# Autodesk Inventor assembly: Montagem1
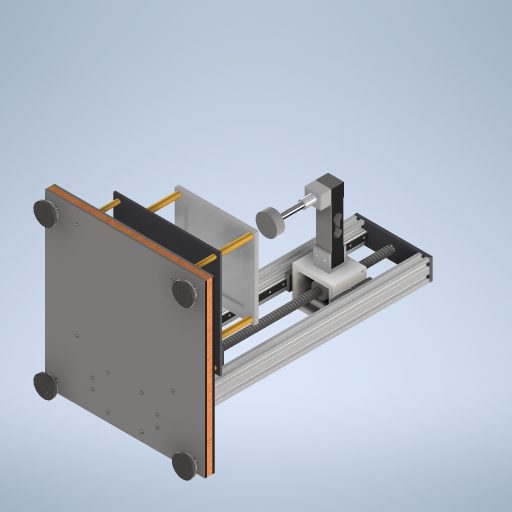
[picture p0: Inventor's stored thumbnail of the model, 512x512]
Saved by Autodesk Inventor 2023 (Build 270158000, 158)
## iProperties
Created: 2023-03-18
Part Number: Montagem1
Document SubType Name: Assembly
Designer: Mateus
Mass: 15449.6 g
Surface Area: 13309.4 cm^2
Volume: 3131.3 cm^3
Density: 4.93393 g/cm^3
Author: Mateus
## Documents named in this file (35)
- C:\Users\Mateus PC\OneDrive\TCC\Desenho 3D\Montagem1.iam
- C:\Users\Mateus PC\OneDrive\TCC\Desenho 3D\Base.ipt
- C:\Users\Mateus PC\OneDrive\TCC\Desenho 3D\Fuso.ipt
- C:\Users\Mateus PC\OneDrive\TCC\Desenho 3D\Motor.ipt
- C:\Users\Mateus PC\OneDrive\TCC\Desenho 3D\Suporte 1.ipt
- C:\Users\Mateus PC\OneDrive\TCC\Desenho 3D\Espaçador 1.ipt
- C:\Users\Mateus PC\OneDrive\TCC\Desenho 3D\Espaçador 2.ipt
- C:\Users\Mateus PC\OneDrive\TCC\Desenho 3D\Suporte 2.ipt
- C:\Users\Mateus PC\OneDrive\TCC\Desenho 3D\Contra ponto.ipt
- C:\Users\Mateus PC\OneDrive\TCC\Desenho 3D\Espaçador 3.ipt
- C:\Users\Mateus PC\OneDrive\TCC\Desenho 3D\Mesa 1.ipt
- C:\Users\Mateus PC\OneDrive\TCC\Desenho 3D\Guia.ipt
- C:\Users\Mateus PC\OneDrive\TCC\Desenho 3D\Suporte guia.ipt
- C:\Users\Mateus PC\OneDrive\TCC\Desenho 3D\Guia trilho.ipt
- C:\Users\Mateus PC\OneDrive\TCC\Desenho 3D\Lado caixa 1.ipt
- C:\Users\Mateus PC\OneDrive\TCC\Desenho 3D\Lado caixa 2.ipt
- C:\Users\Mateus PC\OneDrive\TCC\Desenho 3D\Célula de carga 2.ipt
- C:\Users\Mateus PC\OneDrive\TCC\Desenho 3D\Suporte braço 2.0.ipt
- C:\Users\Mateus PC\OneDrive\TCC\Desenho 3D\Suporte ponta.ipt
- C:\Users\Mateus PC\OneDrive\TCC\Desenho 3D\Trilho 2.ipt
- C:\Users\Mateus PC\OneDrive\TCC\Desenho 3D\Mesa 2.ipt
- C:\Users\Mateus PC\OneDrive\TCC\Desenho 3D\Espaçador 4.ipt
- C:\Users\Mateus PC\OneDrive\TCC\Desenho 3D\Mesa 3.ipt
- C:\Users\Mateus PC\OneDrive\TCC\Desenho 3D\Suporte mesa.ipt
- C:\Users\Mateus PC\OneDrive\TCC\Desenho 3D\Probe.ipt
- C:\Users\Mateus PC\OneDrive\TCC\Desenho 3D\Base madeira.ipt
- C:\Users\Mateus PC\OneDrive\TCC\Desenho 3D\Perfil aluminio 2.ipt
- C:\Users\Mateus PC\OneDrive\TCC\Desenho 3D\Lado caixa 3.ipt
- C:\Users\Mateus PC\OneDrive\TCC\Desenho 3D\Pés.ipt
- C:\Users\Mateus PC\OneDrive\TCC\Desenho 3D\Montagem1\AIP\FEA\eaa23tyn4.fins
- C:\Users\Mateus PC\OneDrive\TCC\Desenho 3D\Montagem1\AIP\FEA\eaa23tyo0.fsat
- C:\Users\Mateus PC\OneDrive\TCC\Desenho 3D\Montagem1\AIP\FEA\eaa23tyo0.ftes
- C:\Users\Mateus PC\OneDrive\TCC\Desenho 3D\Montagem1\AIP\FEA\eaa23tyo0.fwiz
- C:\Users\Mateus PC\OneDrive\TCC\Desenho 3D\Montagem1\AIP\FEA\eaa23tytc.fmsh
- C:\Users\Mateus PC\OneDrive\TCC\Desenho 3D\Montagem1\AIP\FEA\eaa23tytd.fres
## Components (51 placed, 28 different names)
1. Base:1 — Coincidente:13, Alinhado:11, Coincidente:17, Alinhado:12, Coincidente:27, Coincidente:28, Coincidente:29, Coincidente:30, Coincidente:48, Alinhado:28, Alinhado:29, Coincidente:269, Alinhado:84, Coincidente:273, Alinhado:86, Coincidente:275, Flush:104
2. Fuso:1 — Coincidente:9, Coincidente:10, Coincidente:13, Coincidente:49, Coincidente:248, Mate:285
3. Motor:1 — Coincidente:9, Coincidente:10, Alinhado:11, Coincidente:24, Coincidente:25, Coincidente:26, Coincidente:40
4. Suporte 1:1 — Coincidente:24, Coincidente:25, Coincidente:26, Coincidente:31, Coincidente:32, Coincidente:33, Coincidente:34, Coincidente:35, Coincidente:36, Coincidente:37, Coincidente:38, Coincidente:39, Alinhado:22, Mate:117
5. Espaçador 1:1 — Coincidente:29, Coincidente:34, Mate:117
6. Espaçador 1:2 — Coincidente:27, Coincidente:33
7. Espaçador 1:3 — Coincidente:30, Coincidente:32
8. Espaçador 1:4 — Coincidente:28, Coincidente:31
9. Espaçador 2:1 — Coincidente:35, Alinhado:19, Alinhado:20, Coincidente:39, Coincidente:41
10. Espaçador 2:2 — Coincidente:36, Alinhado:20, Alinhado:21
11. Espaçador 2:3 — Coincidente:38, Alinhado:19
12. Espaçador 2:4 — Coincidente:37, Alinhado:21
13. Suporte 2:1 — Coincidente:40, Alinhado:22, Coincidente:41
14. Contra ponto:1 — Coincidente:248, Alinhado:91, Coincidente:278
15. Espaçador 3:1 — Coincidente:45, Alinhado:25, Alinhado:26
16. Espaçador 3:2 — Alinhado:25, Coincidente:47, Coincidente:48, Mate:119
17. Espaçador 3:3 — Coincidente:44, Alinhado:27
18. Espaçador 3:4 — Coincidente:43, Alinhado:26, Alinhado:27
19. Mesa 1:1 — Coincidente:43, Coincidente:44, Coincidente:45, Coincidente:47, Alinhado:28, Alinhado:29, Alinhado:61, Alinhado:62, Mate:119, Mate:121
20. Guia:1 — Coincidente:49, Coincidente:50, Coincidente:51
21. Suporte guia:1 — Coincidente:50, Coincidente:51, Mate:284, Flush:100
22. Guia trilho:1 — Mate:60, Coincidente:206, Alinhado:74
23. Guia trilho:2 — Mate:60, Flush:30, Coincidente:205, Alinhado:74, Alinhado:75, Coincidente:208, Mate:279
24. Guia trilho:3 — Mate:61, Alinhado:72, Alinhado:73
25. Guia trilho:4 — Mate:61, Flush:30, Alinhado:72, Alinhado:73, Coincidente:204, Alinhado:75, Mate:280, Flush:99
26. Lado caixa 1:2 — Mate:115, Flush:65, Coincidente:126, Flush:96, Flush:97, Mate:283
27. Lado caixa 2:2 — Flush:94, Flush:95, Mate:281, Mate:282, Mate:284, Flush:100
28. Célula de carga 2:1 — Coincidente:98, Alinhado:56, Alinhado:57, Flush:63, Flush:64, Mate:114
29. Suporte braço 2.0:1 — Flush:63, Flush:64, Mate:114, Mate:115, Flush:65, Coincidente:126
30. Suporte ponta:1 — Coincidente:98, Alinhado:56, Alinhado:57, Coincidente:270, Coincidente:271
31. Trilho 2:1 — Alinhado:58, Alinhado:59, Coincidente:205, Coincidente:206, Coincidente:208, Coincidente:269, Coincidente:276
32. Trilho 2:2 — Alinhado:58, Alinhado:59, Coincidente:204, Coincidente:277, Alinhado:90
33. Mesa 2:1 — Coincidente:106, Coincidente:107, Coincidente:108, Coincidente:109, Coincidente:110, Alinhado:61, Alinhado:62, Coincidente:111, Coincidente:112, Coincidente:113
34. Espaçador 4:1 — Coincidente:108, Flush:67, Flush:68, Mate:125
35. Espaçador 4:2 — Coincidente:106, Coincidente:110, Flush:68, Mate:123, Mate:124
36. Espaçador 4:3 — Coincidente:109, Flush:66, Flush:67
37. Espaçador 4:4 — Coincidente:107, Flush:66, Mate:122
38. Mesa 3:1 — Coincidente:111, Coincidente:112, Coincidente:113
39. Suporte mesa:1 — Flush:69, Flush:70, Mate:121, Mate:122, Mate:123, Mate:124
40. Suporte mesa:2 — Flush:69, Flush:70, Mate:125
41. Probe:1 — Coincidente:270, Coincidente:271
42. Base madeira:1 — Alinhado:84, Alinhado:85, Coincidente:272, Coincidente:273, Alinhado:86, Alinhado:87, Flush:98
43. Base:2 — Alinhado:85, Coincidente:272, Alinhado:87, Mate:286, Mate:287, Mate:288, Mate:289
44. Perfil aluminio 2:1 — Alinhado:88, Alinhado:89, Coincidente:276, Flush:98, Mate:285
45. Perfil aluminio 2:2 — Alinhado:88, Alinhado:89, Coincidente:275, Coincidente:277, Alinhado:90, Alinhado:91, Coincidente:278
46. Lado caixa 3:1 — Mate:279, Flush:92, Flush:93, Flush:94, Flush:95, Mate:281, Flush:96, Flush:97, Mate:283
47. Lado caixa 3:2 — Mate:280, Flush:92, Flush:93, Mate:282, Flush:99
48. Pés:1 — Mate:287, Flush:102, Flush:103
49. Pés:2 — Mate:288, Flush:101, Flush:102
50. Pés:3 — Mate:286, Flush:103
51. Pés:4 — Mate:289, Flush:101, Flush:104, Mate:290
## Relationships (128: Mate 77, Flush 51)
- Coincidente:9 [Mate] (0.5 mm): Fuso:1 ↔ Motor:1
- Coincidente:10 [Mate]: Fuso:1 ↔ Motor:1
- Coincidente:13 [Mate] (-150 mm): Base:1 ↔ Fuso:1
- Alinhado:11 [Flush] (20 mm): Base:1 ↔ Motor:1
- Coincidente:17 [Mate]: Base:1
- Alinhado:12 [Flush]: Base:1
- Coincidente:24 [Mate]: Motor:1 ↔ Suporte 1:1
- Coincidente:25 [Mate]: Motor:1 ↔ Suporte 1:1
- Coincidente:26 [Mate]: Motor:1 ↔ Suporte 1:1
- Coincidente:27 [Mate]: Base:1 ↔ Espaçador 1:2
- Coincidente:28 [Mate]: Base:1 ↔ Espaçador 1:4
- Coincidente:29 [Mate]: Base:1 ↔ Espaçador 1:1
- Coincidente:30 [Mate]: Base:1 ↔ Espaçador 1:3
- Coincidente:31 [Mate]: Suporte 1:1 ↔ Espaçador 1:4
- Coincidente:32 [Mate]: Suporte 1:1 ↔ Espaçador 1:3
- Coincidente:33 [Mate]: Suporte 1:1 ↔ Espaçador 1:2
- Coincidente:34 [Mate]: Suporte 1:1 ↔ Espaçador 1:1
- Coincidente:35 [Mate]: Suporte 1:1 ↔ Espaçador 2:1
- Coincidente:36 [Mate]: Suporte 1:1 ↔ Espaçador 2:2
- Coincidente:37 [Mate]: Suporte 1:1 ↔ Espaçador 2:4
- Coincidente:38 [Mate]: Suporte 1:1 ↔ Espaçador 2:3
- Alinhado:19 [Flush]: Espaçador 2:1 ↔ Espaçador 2:3
- Alinhado:20 [Flush]: Espaçador 2:1 ↔ Espaçador 2:2
- Alinhado:21 [Flush]: Espaçador 2:2 ↔ Espaçador 2:4
- Coincidente:39 [Mate]: Suporte 1:1 ↔ Espaçador 2:1
- Coincidente:40 [Mate]: Motor:1 ↔ Suporte 2:1
- Alinhado:22 [Flush]: Suporte 1:1 ↔ Suporte 2:1
- Coincidente:41 [Mate]: Espaçador 2:1 ↔ Suporte 2:1
- Coincidente:43 [Mate]: Espaçador 3:4 ↔ Mesa 1:1
- Coincidente:44 [Mate]: Espaçador 3:3 ↔ Mesa 1:1
- Coincidente:45 [Mate]: Espaçador 3:1 ↔ Mesa 1:1
- Alinhado:25 [Flush]: Espaçador 3:1 ↔ Espaçador 3:2
- Alinhado:26 [Flush]: Espaçador 3:1 ↔ Espaçador 3:4
- Alinhado:27 [Flush]: Espaçador 3:3 ↔ Espaçador 3:4
- Coincidente:47 [Mate]: Espaçador 3:2 ↔ Mesa 1:1
- Coincidente:48 [Mate]: Base:1 ↔ Espaçador 3:2
- Alinhado:28 [Flush] (50 mm): Base:1 ↔ Mesa 1:1
- Alinhado:29 [Flush] (18.1 mm): Base:1 ↔ Mesa 1:1
- Coincidente:49 [Mate]: Fuso:1 ↔ Guia:1
- Coincidente:50 [Mate]: Guia:1 ↔ Suporte guia:1
- Coincidente:51 [Mate]: Guia:1 ↔ Suporte guia:1
- Mate:60 (3 mm): Guia trilho:1 ↔ Guia trilho:2
- Mate:61 (3 mm): Guia trilho:3 ↔ Guia trilho:4
- Flush:30: Guia trilho:2 ↔ Guia trilho:4
- Coincidente:98 [Mate]: Célula de carga 2:1 ↔ Suporte ponta:1
- Alinhado:56 [Flush]: Célula de carga 2:1 ↔ Suporte ponta:1
- Alinhado:57 [Flush]: Célula de carga 2:1 ↔ Suporte ponta:1
- Alinhado:58 [Flush]: Trilho 2:1 ↔ Trilho 2:2
- Alinhado:59 [Flush]: Trilho 2:1 ↔ Trilho 2:2
- Coincidente:106 [Mate]: Mesa 2:1 ↔ Espaçador 4:2
- Coincidente:107 [Mate]: Mesa 2:1 ↔ Espaçador 4:4
- Coincidente:108 [Mate]: Mesa 2:1 ↔ Espaçador 4:1
- Coincidente:109 [Mate]: Mesa 2:1 ↔ Espaçador 4:3
- Coincidente:110 [Mate]: Mesa 2:1 ↔ Espaçador 4:2
- Alinhado:61 [Flush] (25 mm): Mesa 1:1 ↔ Mesa 2:1
- Alinhado:62 [Flush] (25 mm): Mesa 1:1 ↔ Mesa 2:1
- Coincidente:111 [Mate]: Mesa 2:1 ↔ Mesa 3:1
- Coincidente:112 [Mate]: Mesa 2:1 ↔ Mesa 3:1
- Coincidente:113 [Mate]: Mesa 2:1 ↔ Mesa 3:1
- Flush:63: Célula de carga 2:1 ↔ Suporte braço 2.0:1
- Flush:64: Célula de carga 2:1 ↔ Suporte braço 2.0:1
- Mate:114: Célula de carga 2:1 ↔ Suporte braço 2.0:1
- Mate:115: Lado caixa 1:2 ↔ Suporte braço 2.0:1
- Flush:65 (15 mm): Lado caixa 1:2 ↔ Suporte braço 2.0:1
- Mate:117: Suporte 1:1 ↔ Espaçador 1:1
- Mate:119: Espaçador 3:2 ↔ Mesa 1:1
- Flush:66: Espaçador 4:3 ↔ Espaçador 4:4
- Flush:67: Espaçador 4:1 ↔ Espaçador 4:3
- Flush:68: Espaçador 4:1 ↔ Espaçador 4:2
- Flush:69: Suporte mesa:1 ↔ Suporte mesa:2
- Flush:70: Suporte mesa:1 ↔ Suporte mesa:2
- Mate:121: Mesa 1:1 ↔ Suporte mesa:1
- Mate:122: Espaçador 4:4 ↔ Suporte mesa:1
- Mate:123: Espaçador 4:2 ↔ Suporte mesa:1
- Mate:124: Espaçador 4:2 ↔ Suporte mesa:1
- Mate:125: Espaçador 4:1 ↔ Suporte mesa:2
- Coincidente:126 [Mate]: Lado caixa 1:2 ↔ Suporte braço 2.0:1
- Alinhado:72 [Flush]: Guia trilho:3 ↔ Guia trilho:4
- Alinhado:73 [Flush]: Guia trilho:3 ↔ Guia trilho:4
- Coincidente:204 [Mate]: Guia trilho:4 ↔ Trilho 2:2
- Coincidente:205 [Mate]: Guia trilho:2 ↔ Trilho 2:1
- Coincidente:206 [Mate]: Guia trilho:1 ↔ Trilho 2:1
- Alinhado:74 [Flush]: Guia trilho:1 ↔ Guia trilho:2
- Alinhado:75 [Flush]: Guia trilho:2 ↔ Guia trilho:4
- Coincidente:208 [Mate]: Guia trilho:2 ↔ Trilho 2:1
- Coincidente:248 [Mate]: Fuso:1 ↔ Contra ponto:1
- Coincidente:269 [Mate] (12.5 mm): Base:1 ↔ Trilho 2:1
- Coincidente:270 [Mate]: Suporte ponta:1 ↔ Probe:1
- Coincidente:271 [Mate] (2 mm): Suporte ponta:1 ↔ Probe:1
- Alinhado:84 [Flush]: Base:1 ↔ Base madeira:1
- Alinhado:85 [Flush]: Base madeira:1 ↔ Base:2
- Coincidente:272 [Mate]: Base madeira:1 ↔ Base:2
- Coincidente:273 [Mate]: Base:1 ↔ Base madeira:1
- Alinhado:86 [Flush]: Base:1 ↔ Base madeira:1
- Alinhado:87 [Flush]: Base madeira:1 ↔ Base:2
- Alinhado:88 [Flush]: Perfil aluminio 2:1 ↔ Perfil aluminio 2:2
- Alinhado:89 [Flush]: Perfil aluminio 2:1 ↔ Perfil aluminio 2:2
- Coincidente:275 [Mate]: Base:1 ↔ Perfil aluminio 2:2
- Coincidente:276 [Mate]: Trilho 2:1 ↔ Perfil aluminio 2:1
- Coincidente:277 [Mate]: Trilho 2:2 ↔ Perfil aluminio 2:2
- Alinhado:90 [Flush] (14 mm): Trilho 2:2 ↔ Perfil aluminio 2:2
- Alinhado:91 [Flush]: Contra ponto:1 ↔ Perfil aluminio 2:2
- Coincidente:278 [Mate]: Contra ponto:1 ↔ Perfil aluminio 2:2
- Mate:279: Guia trilho:2 ↔ Lado caixa 3:1
- Mate:280: Guia trilho:4 ↔ Lado caixa 3:2
- Flush:92: Lado caixa 3:1 ↔ Lado caixa 3:2
- Flush:93: Lado caixa 3:1 ↔ Lado caixa 3:2
- Flush:94: Lado caixa 2:2 ↔ Lado caixa 3:1
- Flush:95: Lado caixa 2:2 ↔ Lado caixa 3:1
- Mate:281: Lado caixa 2:2 ↔ Lado caixa 3:1
- Mate:282: Lado caixa 2:2 ↔ Lado caixa 3:2
- Flush:96: Lado caixa 1:2 ↔ Lado caixa 3:1
- Flush:97: Lado caixa 1:2 ↔ Lado caixa 3:1
- Mate:283: Lado caixa 1:2 ↔ Lado caixa 3:1
- Mate:284: Suporte guia:1 ↔ Lado caixa 2:2
- Flush:98 (28.4 mm): Base madeira:1 ↔ Perfil aluminio 2:1
- Flush:99 (5.25 mm): Guia trilho:4 ↔ Lado caixa 3:2
- Mate:285 (51 mm): Fuso:1 ↔ Perfil aluminio 2:1
- Flush:100 (9.25 mm): Suporte guia:1 ↔ Lado caixa 2:2
- Mate:286: Base:2 ↔ Pés:3
- Mate:287: Base:2 ↔ Pés:1
- Mate:288: Base:2 ↔ Pés:2
- Mate:289: Base:2 ↔ Pés:4
- Flush:101: Pés:2 ↔ Pés:4
- Flush:102: Pés:1 ↔ Pés:2
- Flush:103: Pés:1 ↔ Pés:3
- Flush:104: Base:1 ↔ Pés:4
- Mate:290: Pés:4
## Named parameters: sa_1 = 10000, sa_0 = 10000
note: some values were not read from the file. Shown as the stored number, unit unknown: "sa_1", "sa_0".
